(part 1 of 2)
# Autodesk Inventor assembly: 1000_Planar Winding Jig Overall Assembly_V1
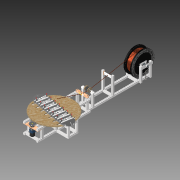
[picture p0: Inventor's stored thumbnail of the model, 180x180]
Saved by Autodesk Inventor 2020 (Build 240168000, 168)
## iProperties
Created: 2019-10-15
Part Number: 1000_Planar Winding Jig Overall Assembly_V1
Document SubType Name: Assembly
Designer: MPI
Author: MPI
## Documents named in this file (59)
- C:\Users\RFLab\Dropbox\MPI Group Folder\Winding Jigs\1000_Planar Winding Jig Overall Assembly_V1.iam
- C:\Users\RFLab\Dropbox\MPI Group Folder\Monika misc\inner winding jig\frame_1385mm.ipt
- C:\Users\RFLab\Dropbox\MPI Group Folder\Monika misc\inner winding jig\frame_1660mm.ipt
- C:\Users\RFLab\Dropbox\MPI Group Folder\Monika misc\inner winding jig\frame_300mm.ipt
- C:\Users\RFLab\Dropbox\MPI Group Folder\Monika misc\inner winding jig\frame_265mm.ipt
- C:\Users\RFLab\Dropbox\MPI Group Folder\Monika misc\inner winding jig\frame_215.5mm.ipt
- C:\Users\RFLab\Dropbox\MPI Group Folder\Monika misc\inner winding jig\frame_210mm.ipt
- C:\Users\RFLab\Dropbox\MPI Group Folder\Monika misc\inner winding jig\frame_275mm.ipt
- C:\Users\RFLab\Dropbox\MPI Group Folder\Monika misc\inner winding jig\frame_318mm.ipt
- C:\Users\RFLab\Dropbox\MPI Group Folder\Monika misc\inner winding jig\frame_440mm.ipt
- C:\Users\RFLab\Dropbox\MPI Group Folder\Monika misc\inner winding jig\frame_370mm.ipt
- C:\Users\RFLab\Dropbox\MPI Group Folder\Monika misc\inner winding jig\92991A190_BRASS CUP POINT SET SCREW.ipt
- C:\Users\RFLab\Dropbox\MPI Group Folder\Winding Jigs\1xxx_Planar Winding Jig\13xx_Winding Former\132x_Former Accessory\1321_Toggle Clamp_V1.ipt
- C:\Users\RFLab\Dropbox\MPI Group Folder\Winding Jigs\1xxx_Planar Winding Jig\13xx_Winding Former\132x_Former Accessory\1322_Clamp Holder_V1.ipt
- C:\Users\RFLab\Dropbox\MPI Group Folder\Winding Jigs\1xxx_Planar Winding Jig\13xx_Winding Former\132x_Former Accessory\1322a_Clamp Holder M4Bolt_V1.ipt
- C:\Users\RFLab\Dropbox\MPI Group Folder\Winding Jigs\1xxx_Planar Winding Jig\13xx_Winding Former\132x_Former Accessory\1323_Clamp Holder Pin_V1.ipt
- C:\Users\RFLab\Documents\Inventor\Content Center Files\R2020\en-US\AS 1474(1)\AS 1474 - M4(1).ipt
- C:\Users\RFLab\Dropbox\MPI Group Folder\Winding Jigs\1xxx_Planar Winding Jig\13xx_Winding Former\132x_Former Accessory\1324_Clamp Rail_V1.ipt
- C:\Users\RFLab\Dropbox\MPI Group Folder\Winding Jigs\1xxx_Planar Winding Jig\13xx_Winding Former\132x_Former Accessory\1325_Former Plate Bolts_V1.ipt
- C:\Users\RFLab\Dropbox\MPI Group Folder\Winding Jigs\1xxx_Planar Winding Jig\13xx_Winding Former\132x_Former Accessory\1326_Thumb Screw_V1.ipt
- C:\Users\RFLab\Dropbox\MPI Group Folder\Winding Jigs\1xxx_Planar Winding Jig\12xx_Non-Frame Structural\122x_Motor and Former Structure\1221_Center Former Shaft_V1.ipt
- C:\Users\RFLab\Dropbox\MPI Group Folder\Winding Jigs\1xxx_Planar Winding Jig\12xx_Non-Frame Structural\122x_Motor and Former Structure\1222_Former Shaft Plate_V1.ipt
- C:\Users\RFLab\Dropbox\MPI Group Folder\Winding Jigs\1xxx_Planar Winding Jig\12xx_Non-Frame Structural\122x_Motor and Former Structure\1223_Motor Plate_V1.ipt
- C:\Users\RFLab\Dropbox\MPI Group Folder\Winding Jigs\1xxx_Planar Winding Jig\12xx_Non-Frame Structural\122x_Motor and Former Structure\1225_Pinon_V1.ipt
- C:\Users\RFLab\Dropbox\MPI Group Folder\Winding Jigs\1xxx_Planar Winding Jig\12xx_Non-Frame Structural\122x_Motor and Former Structure\1225a_Pinion Collar_V1.ipt
- C:\Users\RFLab\Dropbox\MPI Group Folder\Winding Jigs\1xxx_Planar Winding Jig\12xx_Non-Frame Structural\122x_Motor and Former Structure\1226_Flat Head Screw_V1.ipt
- C:\Users\RFLab\Dropbox\MPI Group Folder\Winding Jigs\1xxx_Planar Winding Jig\12xx_Non-Frame Structural\122x_Motor and Former Structure\1224_Stepper Motor_V1.ipt
- C:\Users\RFLab\Dropbox\MPI Group Folder\Winding Jigs\1xxx_Planar Winding Jig\12xx_Non-Frame Structural\122x_Motor and Former Structure\1224a_Stepper Motor Gearbox_V1.ipt
- C:\Users\RFLab\Dropbox\MPI Group Folder\Winding Jigs\1xxx_Planar Winding Jig\13xx_Winding Former\131x_Former Plates\1312_Former Middle_V1.ipt
- C:\Users\RFLab\Dropbox\MPI Group Folder\Winding Jigs\1xxx_Planar Winding Jig\13xx_Winding Former\131x_Former Plates\1311_Former Top_V1.ipt
- C:\Users\RFLab\Dropbox\MPI Group Folder\Winding Jigs\1xxx_Planar Winding Jig\13xx_Winding Former\131x_Former Plates\1313_Former Bottom_V1.ipt
- C:\Users\RFLab\Dropbox\MPI Group Folder\Winding Jigs\1xxx_Planar Winding Jig\12xx_Non-Frame Structural\122x_Motor and Former Structure\1227_Former Shaft Bearing_V1.ipt
- C:\Users\RFLab\Dropbox\MPI Group Folder\Winding Jigs\1xxx_Planar Winding Jig\12xx_Non-Frame Structural\122x_Motor and Former Structure\1228_Major Gear_V1.ipt
- C:\Users\RFLab\Dropbox\MPI Group Folder\Winding Jigs\1xxx_Planar Winding Jig\12xx_Non-Frame Structural\121x_Wire Guidance\1211_Distal Roller Plate_V1.ipt
- C:\Users\RFLab\Dropbox\MPI Group Folder\Winding Jigs\1xxx_Planar Winding Jig\12xx_Non-Frame Structural\121x_Wire Guidance\1212_Roller Plate Bolt_V1.ipt
- C:\Users\RFLab\Dropbox\MPI Group Folder\Winding Jigs\1xxx_Planar Winding Jig\12xx_Non-Frame Structural\121x_Wire Guidance\1213_Distal Roller_V1.ipt
- C:\Users\RFLab\Dropbox\MPI Group Folder\Winding Jigs\1xxx_Planar Winding Jig\12xx_Non-Frame Structural\121x_Wire Guidance\1214_Shaft Collar 3-16_V1.ipt
- C:\Users\RFLab\Dropbox\MPI Group Folder\Winding Jigs\1xxx_Planar Winding Jig\12xx_Non-Frame Structural\121x_Wire Guidance\1215_3-8 Roller Shaft_V1.ipt
- C:\Users\RFLab\Dropbox\MPI Group Folder\Winding Jigs\1xxx_Planar Winding Jig\12xx_Non-Frame Structural\121x_Wire Guidance\1216_Roller Spacer_V1.ipt
- C:\Users\RFLab\Dropbox\MPI Group Folder\Winding Jigs\1xxx_Planar Winding Jig\12xx_Non-Frame Structural\121x_Wire Guidance\1217_17mm Shaft_V1.ipt
- C:\Users\RFLab\Dropbox\MPI Group Folder\Winding Jigs\1xxx_Planar Winding Jig\12xx_Non-Frame Structural\121x_Wire Guidance\1218_Angular Contact Bearing 17mm_V1.ipt
- C:\Users\RFLab\Dropbox\MPI Group Folder\Winding Jigs\1xxx_Planar Winding Jig\12xx_Non-Frame Structural\121x_Wire Guidance\1219_Middle Roller_V1.ipt
- C:\Users\RFLab\Dropbox\MPI Group Folder\Winding Jigs\1xxx_Planar Winding Jig\12xx_Non-Frame Structural\121x_Wire Guidance\12110_Shaft Cap_V1.ipt
- C:\Users\RFLab\Dropbox\MPI Group Folder\Winding Jigs\1xxx_Planar Winding Jig\12xx_Non-Frame Structural\121x_Wire Guidance\12111_Proximal Roller_V1.ipt
- C:\Users\RFLab\Dropbox\MPI Group Folder\Winding Jigs\1xxx_Planar Winding Jig\12xx_Non-Frame Structural\121x_Wire Guidance\12112_Proximal Roller Plate_V1.ipt
- C:\Users\RFLab\Dropbox\MPI Group Folder\Winding Jigs\1xxx_Planar Winding Jig\12xx_Non-Frame Structural\121x_Wire Guidance\12113_Proximal Roller Shaft_V1.ipt
- C:\Users\RFLab\Dropbox\MPI Group Folder\Winding Jigs\1xxx_Planar Winding Jig\12xx_Non-Frame Structural\121x_Wire Guidance\12114_3-8 Shaft Bearing_V1.ipt
- C:\Users\RFLab\Dropbox\MPI Group Folder\Winding Jigs\1xxx_Planar Winding Jig\12xx_Non-Frame Structural\123x_Spool Holder\1231_Spool Shaft_V1.ipt
- C:\Users\RFLab\Dropbox\MPI Group Folder\Winding Jigs\1xxx_Planar Winding Jig\12xx_Non-Frame Structural\123x_Spool Holder\1233_Spool Holding Bolts_V1.ipt
- C:\Users\RFLab\Dropbox\MPI Group Folder\Winding Jigs\1xxx_Planar Winding Jig\12xx_Non-Frame Structural\123x_Spool Holder\1232_Spool Shaft Collar_V1.ipt
- C:\Users\RFLab\Dropbox\MPI Group Folder\Winding Jigs\1xxx_Planar Winding Jig\12xx_Non-Frame Structural\123x_Spool Holder\1234_Spool Plate_V1.ipt
- C:\Users\RFLab\Dropbox\MPI Group Folder\Winding Jigs\1xxx_Planar Winding Jig\12xx_Non-Frame Structural\123x_Spool Holder\1235_Shaft Locking Screw_V1.ipt
- C:\Users\RFLab\Dropbox\MPI Group Folder\Winding Jigs\1xxx_Planar Winding Jig\12xx_Non-Frame Structural\123x_Spool Holder\1236_Spool Shaft Support Plate_V1.ipt
- C:\Users\RFLab\Dropbox\MPI Group Folder\Winding Jigs\1xxx_Planar Winding Jig\12xx_Non-Frame Structural\123x_Spool Holder\1237_Turnbuckle_V1.ipt
- C:\Users\RFLab\Dropbox\MPI Group Folder\Winding Jigs\1xxx_Planar Winding Jig\12xx_Non-Frame Structural\123x_Spool Holder\1238_Hex Nut Turnbuckle_V1.ipt
- C:\Users\RFLab\Dropbox\MPI Group Folder\Winding Jigs\1xxx_Planar Winding Jig\12xx_Non-Frame Structural\123x_Spool Holder\1239_Turnbuckle Holding Bolt_V1.ipt
- C:\Users\RFLab\Dropbox\MPI Group Folder\Winding Jigs\1xxx_Planar Winding Jig\12xx_Non-Frame Structural\123x_Spool Holder\12310_Washer_V1.ipt
- C:\Users\RFLab\Dropbox\MPI Group Folder\Winding Jigs\1xxx_Planar Winding Jig\12xx_Non-Frame Structural\1240_Wire Spool and Wire.ipt
- C:\Users\RFLab\Dropbox\MPI Group Folder\Winding Jigs\1xxx_Planar Winding Jig\12xx_Non-Frame Structural\1240x_Wire Depiction_V1.ipt
## Components (321 placed, 58 different names)
1. 1222_Former Shaft Plate_V1:1 — Mate:46, Flush:77, Mate:47, Insert:1
2. 1222_Former Shaft Plate_V1:2 — Mate:48, Flush:78, Mate:49
3. 1221_Center Former Shaft_V1:1 — Insert:1, Mate:51, Mate:53, Mate:55, Mate:57
4. 1228_Major Gear_V1:1 — Mate:50, Mate:51, Insert:2, Mate:52, Insert:3, Insert:4, Insert:5, Insert:6, Insert:7, Insert:8, Insert:9, Insert:10, Insert:11, Insert:12, Insert:13, Insert:14, Insert:15, Insert:16, Flush:84
5. 1227_Former Shaft Bearing_V1:1 — Insert:2
6. 1224a_Stepper Motor Gearbox_V1:1 — Insert:38, Insert:39, Insert:40, Insert:41, Mate:65
7. 1224_Stepper Motor_V1:1 — Insert:40, Insert:41
8. 1225_Pinon_V1:1 — Flush:84, Mate:64, Insert:42, Insert:43
9. 1225a_Pinion Collar_V1:1 — Mate:64, Mate:65, Insert:42, Insert:43, Angle:36
10. 1211_Distal Roller Plate_V1:1 — Insert:46, Insert:47, Flush:87, Flush:88, Insert:50, Insert:51, Insert:58, Insert:59, Mate:70, Mate:72
11. 1213_Distal Roller_V1:1 — Insert:44, Insert:46, Insert:48
12. 1213_Distal Roller_V1:2 — Insert:45, Insert:47, Insert:49, Mate:68, Flush:294
13. 12114_3-8 Shaft Bearing_V1:1 — Insert:44
14. 12114_3-8 Shaft Bearing_V1:2 — Insert:45
15. 12114_3-8 Shaft Bearing_V1:3 — Insert:48
16. 12114_3-8 Shaft Bearing_V1:4 — Insert:49
17. 1211_Distal Roller Plate_V1:2 — Mate:68, Flush:87, Flush:88, Insert:52, Insert:53, Insert:54, Insert:55, Insert:56, Insert:57
18. 1216_Roller Spacer_V1:1 — Insert:51
19. 1216_Roller Spacer_V1:2 — Insert:50
20. 1212_Roller Plate Bolt_V1:1 — Insert:52
21. 1212_Roller Plate Bolt_V1:2 — Insert:53
22. 1215_3-8 Roller Shaft_V1:1 — Insert:54
23. 1215_3-8 Roller Shaft_V1:2 — Insert:55
24. 1214_Shaft Collar 3-16_V1:1 — Insert:58
25. 1214_Shaft Collar 3-16_V1:2 — Insert:59
26. 1214_Shaft Collar 3-16_V1:3 — Insert:56
27. 1214_Shaft Collar 3-16_V1:4 — Insert:57
28. 12110_Shaft Cap_V1:1 — Mate:75, Mate:76, Mate:77
29. 12110_Shaft Cap_V1:2 — Mate:78, Mate:79, Mate:80, Insert:60, Insert:61
30. 1219_Middle Roller_V1:1 — Insert:61, Insert:62, Insert:63, Flush:292
31. 1217_17mm Shaft_V1:1 — Insert:60
32. 1218_Angular Contact Bearing 17mm_V1:1 — Insert:62
33. 1218_Angular Contact Bearing 17mm_V1:2 — Insert:63
34. frame_440mm:1 — Mate:81, Flush:97, Flush:98, Mate:84, Flush:103, Flush:104
35. frame_440mm:2 — Mate:82, Flush:99, Flush:100, Mate:83, Flush:101, Flush:102
36. 12112_Proximal Roller Plate_V1:1 — Mate:83, Flush:101, Flush:102, Insert:74, Insert:75
37. 12112_Proximal Roller Plate_V1:2 — Mate:84, Flush:103, Flush:104, Insert:64, Insert:65, Insert:70, Insert:71, Insert:72, Insert:73
38. 12113_Proximal Roller Shaft_V1:1 — Insert:64
39. 12113_Proximal Roller Shaft_V1:2 — Insert:65
40. 12111_Proximal Roller_V1:1 — Insert:66, Insert:68, Insert:70
41. 12111_Proximal Roller_V1:2 — Insert:67, Insert:69, Insert:71
42. 12114_3-8 Shaft Bearing_V1:5 — Insert:66
43. 12114_3-8 Shaft Bearing_V1:6 — Insert:68
44. 12114_3-8 Shaft Bearing_V1:7 — Insert:67
45. 12114_3-8 Shaft Bearing_V1:8 — Insert:69
46. 1236_Spool Shaft Support Plate_V1:1 — Mate:90, Flush:114, Flush:115, Flush:116, Insert:76, Insert:77, Angle:37
47. 1236_Spool Shaft Support Plate_V1:2 — Mate:89, Flush:111, Flush:112, Flush:113, Insert:78, Angle:1
48. 92991A190_BRASS CUP POINT SET SCREW:1 — Insert:73
49. 92991A190_BRASS CUP POINT SET SCREW:2 — Insert:72
50. 92991A190_BRASS CUP POINT SET SCREW:3 — Insert:75
51. 92991A190_BRASS CUP POINT SET SCREW:4 — Insert:74
52. 1231_Spool Shaft_V1:1 — Insert:76, Angle:1, Mate:354, Mate:360
53. 1232_Spool Shaft Collar_V1:1 — Insert:77
54. 1232_Spool Shaft Collar_V1:2 — Insert:78
55. 1240_Wire Spool and Wire:1 — Mate:354, Mate:355, Mate:356, Angle:34, Flush:292, Mate:357, Mate:358, Mate:359
56. 1234_Spool Plate_V1:1 — Insert:84, Insert:85, Insert:86, Mate:355, Flush:293, Angle:37, Flush:295, Flush:296, Mate:360
57. 1234_Spool Plate_V1:2 — Insert:82, Insert:83, Insert:87, Mate:356, Angle:34, Flush:293, Flush:295, Flush:296
58. 1233_Spool Holding Bolts_V1:1 — Insert:82
59. 1233_Spool Holding Bolts_V1:2 — Insert:83
60. 1233_Spool Holding Bolts_V1:3 — Insert:84
61. 1233_Spool Holding Bolts_V1:4 — Insert:85
62. 1235_Shaft Locking Screw_V1:1 — Insert:86
63. 1235_Shaft Locking Screw_V1:2 — Insert:87
64. 12310_Washer_V1:1 — Insert:88, Insert:91
65. 12310_Washer_V1:2 — Insert:89, Insert:90
66. 1239_Turnbuckle Holding Bolt_V1:1 — Insert:91, Mate:91, Insert:98
67. 1239_Turnbuckle Holding Bolt_V1:2 — Insert:90, Mate:92, Insert:99
68. 12310_Washer_V1:3 — Insert:92, Insert:96
69. 12310_Washer_V1:4 — Insert:93, Insert:94
70. 1238_Hex Nut Turnbuckle_V1:1 — Insert:94, Insert:95
71. 1238_Hex Nut Turnbuckle_V1:2 — Insert:95
72. 1238_Hex Nut Turnbuckle_V1:3 — Insert:96, Insert:97
73. 1238_Hex Nut Turnbuckle_V1:4 — Insert:97
74. 1237_Turnbuckle_V1:1 — Mate:91, Angle:3
75. 1237_Turnbuckle_V1:2 — Mate:92, Angle:4
76. 1238_Hex Nut Turnbuckle_V1:5 — Insert:98
77. 1238_Hex Nut Turnbuckle_V1:6 — Insert:99
78. 1240x_Wire Depiction_V1:1 — Mate:357, Mate:358, Angle:35, Mate:359, Flush:294
79. frame_318mm:2 — Mate:74, Flush:95, Flush:96, Mate:75, Mate:76, Mate:77
80. frame_318mm:1 — Mate:73, Flush:93, Flush:94, Mate:78, Mate:79, Mate:80
81. frame_275mm:2 — Mate:71, Mate:72, Flush:91, Flush:92
82. frame_275mm:1 — Mate:69, Mate:70, Flush:89, Flush:90
83. frame_370mm:4 — Flush:107, Mate:86, Flush:116, Angle:4
84. frame_370mm:3 — Flush:105, Flush:106, Mate:85, Mate:90, Flush:114, Flush:115
85. frame_370mm:2 — Mate:88, Flush:110, Flush:113, Angle:3
86. frame_370mm:1 — Mate:87, Flush:108, Flush:109, Mate:89, Flush:111, Flush:112
87. frame_1385mm:1 — Mate:1, Flush:1, Mate:2, Flush:2, Flush:3, Mate:3, Mate:9, Mate:10, Flush:18, Mate:14, Flush:20, Mate:15, Mate:22, Flush:34, Mate:23, Flush:36, Mate:24, Flush:38, Flush:46, Flush:47, Flush:67, Mate:38, Mate:39
88. frame_1385mm:2 — Flush:2, Flush:3, Mate:3, Flush:4, Mate:4, Mate:5, Flush:6, Mate:8, Flush:7, Flush:8, Flush:9, Flush:10, Flush:11, Flush:12, Mate:11, Flush:13, Flush:14, Mate:12, Flush:15, Mate:19, Flush:28, Mate:20, Flush:30, Mate:21, Flush:32, Flush:33, Flush:44, Flush:45, Mate:47
89. frame_1660mm:2 — Flush:4, Mate:4, Mate:5, Flush:66, Flush:74, Mate:69, Flush:90, Mate:74, Flush:96, Mate:82, Flush:99, Mate:87, Mate:88, Flush:108, Flush:109, Flush:110, Insert:88, Insert:92
90. frame_300mm:1 — Flush:6, Mate:8, Flush:7
91. frame_300mm:2 — Flush:8, Mate:9, Flush:9, Flush:61, Mate:46, Flush:77
92. frame_300mm:3 — Flush:10, Mate:10, Flush:11, Flush:63
93. frame_265mm:1 — Flush:12, Mate:11, Flush:13, Mate:13, Flush:17, Flush:19, Flush:29
94. frame_265mm:2 — Flush:14, Mate:12, Flush:15, Flush:16, Flush:21, Flush:31
95. frame_265mm:3 — Flush:16, Mate:13, Flush:17, Mate:17, Flush:24, Flush:25, Mate:18, Flush:26, Flush:27
96. frame_265mm:4 — Flush:18, Mate:14, Flush:19, Flush:22, Mate:16, Flush:23, Flush:37
97. frame_265mm:5 — Flush:20, Mate:15, Flush:21, Flush:39, Flush:42
98. frame_265mm:6 — Flush:22, Mate:16, Flush:23, Mate:25, Flush:40, Flush:41, Mate:26, Flush:43
99. frame_215.5mm:1 — Mate:19, Flush:28, Flush:29
100. frame_215.5mm:2 — Mate:20, Flush:30, Flush:31
101. frame_215.5mm:3 — Mate:17, Flush:24, Flush:25
102. frame_215.5mm:4 — Mate:18, Flush:26, Flush:27, Mate:32, Flush:54, Flush:55
103. frame_215.5mm:5 — Mate:21, Flush:32, Flush:33, Flush:35, Mate:27
104. frame_215.5mm:6 — Mate:25, Flush:40, Flush:41, Mate:29, Flush:48, Flush:49
105. frame_215.5mm:7 — Mate:24, Flush:38, Flush:39
106. frame_215.5mm:8 — Mate:22, Flush:34, Flush:35, Mate:28
107. frame_215.5mm:9 — Mate:23, Flush:36, Flush:37
108. frame_215.5mm:10 — Mate:26, Flush:42, Flush:43
109. frame_1385mm:3 — Mate:27, Flush:44, Flush:45, Mate:33, Mate:34, Mate:49, Mate:63, Flush:82, Flush:83
110. frame_1385mm:4 — Mate:28, Flush:46, Flush:47, Mate:30, Mate:31, Mate:35, Flush:60, Mate:36, Flush:62, Mate:50, Angle:9, Angle:36
111. frame_265mm:7 — Mate:29, Flush:48, Flush:49, Flush:50, Flush:51, Flush:52, Flush:53
112. frame_265mm:8 — Mate:31, Flush:52, Flush:53
113. frame_265mm:9 — Mate:32, Flush:54, Flush:55, Flush:56, Flush:57, Flush:58, Flush:59
114. frame_265mm:10 — Mate:30, Flush:50, Flush:51
115. frame_265mm:11 — Mate:34, Flush:58, Flush:59
116. frame_265mm:12 — Mate:33, Flush:56, Flush:57
117. frame_300mm:4 — Mate:35, Flush:60, Flush:61, Mate:48, Flush:78
118. frame_300mm:5 — Mate:36, Flush:62, Flush:63
119. frame_210mm:1 — Mate:40, Flush:68, Flush:69, Mate:43, Flush:76, Flush:89, Flush:91
120. frame_210mm:2 — Mate:42, Flush:72, Mate:43, Flush:93, Flush:95
121. frame_210mm:3 — Mate:44, Flush:73, Flush:74, Flush:98, Flush:100
122. frame_210mm:4 — Mate:45, Flush:75, Flush:76
123. frame_1660mm:3 — Flush:66, Flush:67, Mate:38, Mate:39, Mate:40, Flush:68, Flush:69, Mate:42, Flush:72, Mate:44, Flush:73, Mate:45, Flush:75, Mate:71, Flush:92, Mate:73, Flush:94, Mate:81, Flush:97, Flush:105, Flush:106, Mate:85, Flush:107, Mate:86, Insert:89, Insert:93
124. 1325_Former Plate Bolts_V1:1 — Insert:100
125. 1325_Former Plate Bolts_V1:2 — Insert:101
126. 1325_Former Plate Bolts_V1:3 — Insert:102
127. 1325_Former Plate Bolts_V1:4 — Insert:103
128. 1325_Former Plate Bolts_V1:5 — Insert:104
129. 1325_Former Plate Bolts_V1:6 — Insert:105
130. 1325_Former Plate Bolts_V1:7 — Insert:106
131. 1325_Former Plate Bolts_V1:8 — Insert:107
132. 1325_Former Plate Bolts_V1:9 — Insert:108
133. 1325_Former Plate Bolts_V1:10 — Insert:109
134. 1325_Former Plate Bolts_V1:11 — Insert:110
135. 1325_Former Plate Bolts_V1:12 — Insert:111
136. 1313_Former Bottom_V1:1 — Mate:52, Mate:53, Insert:3, Insert:4, Mate:54, Insert:17, Angle:9
137. 1226_Flat Head Screw_V1:1 — Insert:10
138. 1226_Flat Head Screw_V1:2 — Insert:14
139. 1226_Flat Head Screw_V1:3 — Insert:15
140. 1226_Flat Head Screw_V1:4 — Insert:7
141. 1226_Flat Head Screw_V1:5 — Insert:11
142. 1226_Flat Head Screw_V1:6 — Insert:12
143. 1226_Flat Head Screw_V1:7 — Insert:13
144. 1226_Flat Head Screw_V1:8 — Insert:5
145. 1226_Flat Head Screw_V1:9 — Insert:16
146. 1226_Flat Head Screw_V1:10 — Insert:9
147. 1226_Flat Head Screw_V1:11 — Insert:8
148. 1226_Flat Head Screw_V1:12 — Insert:6
149. 1312_Former Middle_V1:1 — Mate:54, Mate:55, Insert:17, Mate:56, Insert:18
150. 1311_Former Top_V1:1 — Mate:56, Mate:57, Insert:18, Mate:58, Insert:31, Insert:32, Mate:59, Insert:33, Insert:34, Mate:60, Insert:35, Insert:36, Insert:37, Insert:100, Insert:101, Insert:102, Insert:103, Insert:104, Insert:105, Insert:106, Insert:107, Insert:108, Insert:109, Insert:110, Insert:111, Mate:122, Flush:134, Mate:160, Mate:163, Mate:164, Flush:160, Mate:201, Mate:202, Mate:203, Mate:348, Mate:349, Mate:350, Mate:351, Mate:352, Mate:353
151. 1326_Thumb Screw_V1:1 — Insert:37
152. 1326_Thumb Screw_V1:2 — Insert:36
153. 1223_Motor Plate_V1:1 — Mate:63, Flush:82, Flush:83, Insert:38, Insert:39
154. 1324_Clamp Rail_V1:1 — Mate:58, Insert:31, Insert:32, Flush:79
155. 1324_Clamp Rail_V1:2 — Mate:59, Insert:33, Insert:34, Mate:61, Mate:123, Flush:135
156. 1322_Clamp Holder_V1:1 — Mate:60, Flush:79, Mate:61, Mate:62, Flush:80, Flush:81, Mate:93, Mate:94, Angle:5, Mate:95, Mate:96, Angle:6, Mate:97, Mate:98, Mate:99, Mate:125
157. 1321_Toggle Clamp_V1:1 — Mate:62, Flush:80, Flush:81, Mate:101, Mate:103, Mate:105
158. 1323_Clamp Holder Pin_V1:1 — Insert:35, Mate:125
159. BS 3692 Precision hexagon bolts and screws (Full Threaded) - Metric M4 x 9:1 — Mate:95, Mate:96, Angle:6, Flush:119, Mate:100
160. BS 3692 Precision hexagon bolts and screws (Full Threaded) - Metric M4 x 9:2 — Mate:93, Mate:94, Angle:5, Flush:120, Mate:106
161. BS 3692 Precision hexagon bolts and screws (Full Threaded) - Metric M4 x 9:3 — Flush:118, Mate:99, Flush:120, Mate:104
162. BS 3692 Precision hexagon bolts and screws (Full Threaded) - Metric M4 x 9:4 — Flush:118, Mate:97, Mate:98, Flush:119, Mate:102
163. AS 1474 - Metric M4:1 — Mate:100, Mate:101, Flush:124
164. AS 1474 - Metric M4:2 — Flush:121, Flush:123, Mate:102, Mate:103
165. AS 1474 - Metric M4:3 — Flush:122, Flush:123, Mate:104
166. AS 1474 - Metric M4:4 — Flush:121, Flush:122, Mate:105, Mate:106, Flush:124
167. 1322_Clamp Holder_V1:2 — Mate:122, Mate:123, Mate:124, Flush:135
168. 1321_Toggle Clamp_V1:2
169. 1323_Clamp Holder Pin_V1:2 — Flush:134, Mate:124, Flush:185
170. BS 3692 Precision hexagon bolts and screws (Full Threaded) - Metric M4 x 9:5
171. BS 3692 Precision hexagon bolts and screws (Full Threaded) - Metric M4 x 9:6
172. BS 3692 Precision hexagon bolts and screws (Full Threaded) - Metric M4 x 9:7
173. BS 3692 Precision hexagon bolts and screws (Full Threaded) - Metric M4 x 9:8
174. AS 1474 - Metric M4:5
175. AS 1474 - Metric M4:6
176. AS 1474 - Metric M4:7
177. AS 1474 - Metric M4:8
178. 1324_Clamp Rail_V1:3 — Mate:160, Flush:156, Mate:162, Flush:158
179. 1324_Clamp Rail_V1:4 — Flush:156, Mate:161, Mate:163, Mate:164, Flush:158
180. 1322_Clamp Holder_V1:3 — Mate:161, Flush:157
181. 1321_Toggle Clamp_V1:3
182. 1323_Clamp Holder Pin_V1:3 — Flush:159
183. BS 3692 Precision hexagon bolts and screws (Full Threaded) - Metric M4 x 9:9
184. BS 3692 Precision hexagon bolts and screws (Full Threaded) - Metric M4 x 9:10
185. BS 3692 Precision hexagon bolts and screws (Full Threaded) - Metric M4 x 9:11
186. BS 3692 Precision hexagon bolts and screws (Full Threaded) - Metric M4 x 9:12
187. AS 1474 - Metric M4:9
188. AS 1474 - Metric M4:10
189. AS 1474 - Metric M4:11
190. AS 1474 - Metric M4:12
191. 1322_Clamp Holder_V1:4 — Flush:157, Mate:162
192. 1321_Toggle Clamp_V1:4
193. 1323_Clamp Holder Pin_V1:4 — Flush:159, Flush:160, Flush:291
194. BS 3692 Precision hexagon bolts and screws (Full Threaded) - Metric M4 x 9:13
195. BS 3692 Precision hexagon bolts and screws (Full Threaded) - Metric M4 x 9:14
196. BS 3692 Precision hexagon bolts and screws (Full Threaded) - Metric M4 x 9:15
197. BS 3692 Precision hexagon bolts and screws (Full Threaded) - Metric M4 x 9:16
198. AS 1474 - Metric M4:13
199. AS 1474 - Metric M4:14
200. AS 1474 - Metric M4:15
201. AS 1474 - Metric M4:16
202. 1324_Clamp Rail_V1:5
203. 1324_Clamp Rail_V1:6 — Mate:201, Mate:202, Mate:203
204. 1322_Clamp Holder_V1:5
205. 1321_Toggle Clamp_V1:5
206. 1323_Clamp Holder Pin_V1:5
207. BS 3692 Precision hexagon bolts and screws (Full Threaded) - Metric M4 x 9:17
208. BS 3692 Precision hexagon bolts and screws (Full Threaded) - Metric M4 x 9:18
209. BS 3692 Precision hexagon bolts and screws (Full Threaded) - Metric M4 x 9:19
210. BS 3692 Precision hexagon bolts and screws (Full Threaded) - Metric M4 x 9:20
211. AS 1474 - Metric M4:17
212. AS 1474 - Metric M4:18
213. AS 1474 - Metric M4:19
214. AS 1474 - Metric M4:20
215. 1322_Clamp Holder_V1:6
216. 1321_Toggle Clamp_V1:6
217. 1323_Clamp Holder Pin_V1:6 — Flush:185
218. BS 3692 Precision hexagon bolts and screws (Full Threaded) - Metric M4 x 9:21
219. BS 3692 Precision hexagon bolts and screws (Full Threaded) - Metric M4 x 9:22
220. BS 3692 Precision hexagon bolts and screws (Full Threaded) - Metric M4 x 9:23
221. BS 3692 Precision hexagon bolts and screws (Full Threaded) - Metric M4 x 9:24
222. AS 1474 - Metric M4:21
223. AS 1474 - Metric M4:22
224. AS 1474 - Metric M4:23
225. AS 1474 - Metric M4:24
226. 1324_Clamp Rail_V1:7 — Flush:282, Flush:285
227. 1324_Clamp Rail_V1:8 — Mate:348, Mate:349, Mate:350
228. 1322_Clamp Holder_V1:7
229. 1321_Toggle Clamp_V1:7
230. 1323_Clamp Holder Pin_V1:7
231. BS 3692 Precision hexagon bolts and screws (Full Threaded) - Metric M4 x 9:25
232. BS 3692 Precision hexagon bolts and screws (Full Threaded) - Metric M4 x 9:26
233. BS 3692 Precision hexagon bolts and screws (Full Threaded) - Metric M4 x 9:27
234. BS 3692 Precision hexagon bolts and screws (Full Threaded) - Metric M4 x 9:28
235. AS 1474 - Metric M4:25
236. AS 1474 - Metric M4:26
237. AS 1474 - Metric M4:27
238. AS 1474 - Metric M4:28
239. 1322_Clamp Holder_V1:8
240. 1321_Toggle Clamp_V1:8
241. 1323_Clamp Holder Pin_V1:8 — Flush:288, Flush:291
242. BS 3692 Precision hexagon bolts and screws (Full Threaded) - Metric M4 x 9:29
243. BS 3692 Precision hexagon bolts and screws (Full Threaded) - Metric M4 x 9:30
244. BS 3692 Precision hexagon bolts and screws (Full Threaded) - Metric M4 x 9:31
245. BS 3692 Precision hexagon bolts and screws (Full Threaded) - Metric M4 x 9:32
246. AS 1474 - Metric M4:29
247. AS 1474 - Metric M4:30
248. AS 1474 - Metric M4:31
249. AS 1474 - Metric M4:32
250. 1324_Clamp Rail_V1:9 — Flush:286, Mate:351
251. 1324_Clamp Rail_V1:10 — Flush:282, Flush:283, Flush:285
252. 1322_Clamp Holder_V1:9
253. 1321_Toggle Clamp_V1:9
254. 1323_Clamp Holder Pin_V1:9
255. BS 3692 Precision hexagon bolts and screws (Full Threaded) - Metric M4 x 9:33
256. BS 3692 Precision hexagon bolts and screws (Full Threaded) - Metric M4 x 9:34
257. BS 3692 Precision hexagon bolts and screws (Full Threaded) - Metric M4 x 9:35
258. BS 3692 Precision hexagon bolts and screws (Full Threaded) - Metric M4 x 9:36
259. AS 1474 - Metric M4:33
260. AS 1474 - Metric M4:34
261. AS 1474 - Metric M4:35
262. AS 1474 - Metric M4:36
263. 1322_Clamp Holder_V1:10
264. 1321_Toggle Clamp_V1:10
265. 1323_Clamp Holder Pin_V1:10 — Flush:288, Flush:289
266. BS 3692 Precision hexagon bolts and screws (Full Threaded) - Metric M4 x 9:37
267. BS 3692 Precision hexagon bolts and screws (Full Threaded) - Metric M4 x 9:38
268. BS 3692 Precision hexagon bolts and screws (Full Threaded) - Metric M4 x 9:39
269. BS 3692 Precision hexagon bolts and screws (Full Threaded) - Metric M4 x 9:40
270. AS 1474 - Metric M4:37
271. AS 1474 - Metric M4:38
272. AS 1474 - Metric M4:39
273. AS 1474 - Metric M4:40
274. 1324_Clamp Rail_V1:11 — Flush:284, Flush:287
275. 1324_Clamp Rail_V1:12 — Flush:283, Flush:286, Mate:352
276. 1322_Clamp Holder_V1:11
277. 1321_Toggle Clamp_V1:11
278. 1323_Clamp Holder Pin_V1:11
279. BS 3692 Precision hexagon bolts and screws (Full Threaded) - Metric M4 x 9:41
280. BS 3692 Precision hexagon bolts and screws (Full Threaded) - Metric M4 x 9:42
281. BS 3692 Precision hexagon bolts and screws (Full Threaded) - Metric M4 x 9:43
282. BS 3692 Precision hexagon bolts and screws (Full Threaded) - Metric M4 x 9:44
283. AS 1474 - Metric M4:41
284. AS 1474 - Metric M4:42
285. AS 1474 - Metric M4:43
286. AS 1474 - Metric M4:44
287. 1322_Clamp Holder_V1:12
288. 1321_Toggle Clamp_V1:12
289. 1323_Clamp Holder Pin_V1:12 — Flush:289, Flush:290
290. BS 3692 Precision hexagon bolts and screws (Full Threaded) - Metric M4 x 9:45
291. BS 3692 Precision hexagon bolts and screws (Full Threaded) - Metric M4 x 9:46
292. BS 3692 Precision hexagon bolts and screws (Full Threaded) - Metric M4 x 9:47
293. BS 3692 Precision hexagon bolts and screws (Full Threaded) - Metric M4 x 9:48
294. AS 1474 - Metric M4:45
295. AS 1474 - Metric M4:46
296. AS 1474 - Metric M4:47
297. AS 1474 - Metric M4:48
298. 1324_Clamp Rail_V1:13
299. 1324_Clamp Rail_V1:14 — Flush:284, Flush:287, Mate:353
300. 1322_Clamp Holder_V1:13
301. 1321_Toggle Clamp_V1:13
302. 1323_Clamp Holder Pin_V1:13
303. BS 3692 Precision hexagon bolts and screws (Full Threaded) - Metric M4 x 9:49
304. BS 3692 Precision hexagon bolts and screws (Full Threaded) - Metric M4 x 9:50
305. BS 3692 Precision hexagon bolts and screws (Full Threaded) - Metric M4 x 9:51
306. BS 3692 Precision hexagon bolts and screws (Full Threaded) - Metric M4 x 9:52
307. AS 1474 - Metric M4:49
308. AS 1474 - Metric M4:50
309. AS 1474 - Metric M4:51
310. AS 1474 - Metric M4:52
311. 1322_Clamp Holder_V1:14
312. 1321_Toggle Clamp_V1:14
313. 1323_Clamp Holder Pin_V1:14 — Flush:290
314. BS 3692 Precision hexagon bolts and screws (Full Threaded) - Metric M4 x 9:53
315. BS 3692 Precision hexagon bolts and screws (Full Threaded) - Metric M4 x 9:54
316. BS 3692 Precision hexagon bolts and screws (Full Threaded) - Metric M4 x 9:55
317. BS 3692 Precision hexagon bolts and screws (Full Threaded) - Metric M4 x 9:56
318. AS 1474 - Metric M4:53
319. AS 1474 - Metric M4:54
320. AS 1474 - Metric M4:55
321. AS 1474 - Metric M4:56
## Relationships (774: Mate 354, Flush 288, Insert 96, Angle 36)
- Mate:1: frame_1385mm:1
- Flush:1: frame_1385mm:1
- Mate:2: frame_1385mm:1
- Flush:2: frame_1385mm:1 ↔ frame_1385mm:2
- Flush:3: frame_1385mm:1 ↔ frame_1385mm:2
- Mate:3 (300 mm): frame_1385mm:1 ↔ frame_1385mm:2
- Flush:4: frame_1385mm:2 ↔ frame_1660mm:2
- Mate:4: frame_1385mm:2 ↔ frame_1660mm:2
- Mate:5 (-45 mm): frame_1385mm:2 ↔ frame_1660mm:2
- Flush:6: frame_1385mm:2 ↔ frame_300mm:1
- Mate:8: frame_1385mm:2 ↔ frame_300mm:1
- Flush:7 (27 mm): frame_1385mm:2 ↔ frame_300mm:1
- Flush:8: frame_1385mm:2 ↔ frame_300mm:2
- Mate:9: frame_1385mm:1 ↔ frame_300mm:2
- Flush:9 (537 mm): frame_1385mm:2 ↔ frame_300mm:2
- Flush:10: frame_1385mm:2 ↔ frame_300mm:3
- Mate:10: frame_1385mm:1 ↔ frame_300mm:3
- Flush:11 (657 mm): frame_1385mm:2 ↔ frame_300mm:3
- Flush:12: frame_1385mm:2 ↔ frame_265mm:1
- Mate:11: frame_1385mm:2 ↔ frame_265mm:1
- Flush:13 (487 mm): frame_1385mm:2 ↔ frame_265mm:1
- Flush:14: frame_1385mm:2 ↔ frame_265mm:2
- Mate:12: frame_1385mm:2 ↔ frame_265mm:2
- Flush:15 (707 mm): frame_1385mm:2 ↔ frame_265mm:2
- Flush:16: frame_265mm:2 ↔ frame_265mm:3
- Mate:13: frame_265mm:1 ↔ frame_265mm:3
- Flush:17: frame_265mm:1 ↔ frame_265mm:3
- Flush:18: frame_1385mm:1 ↔ frame_265mm:4
- Mate:14: frame_1385mm:1 ↔ frame_265mm:4
- Flush:19: frame_265mm:1 ↔ frame_265mm:4
- Flush:20: frame_1385mm:1 ↔ frame_265mm:5
- Mate:15: frame_1385mm:1 ↔ frame_265mm:5
- Flush:21: frame_265mm:2 ↔ frame_265mm:5
- Flush:22: frame_265mm:4 ↔ frame_265mm:6
- Mate:16: frame_265mm:4 ↔ frame_265mm:6
- Flush:23: frame_265mm:4 ↔ frame_265mm:6
- Mate:17: frame_265mm:3 ↔ frame_215.5mm:3
- Flush:24: frame_265mm:3 ↔ frame_215.5mm:3
- Flush:25: frame_265mm:3 ↔ frame_215.5mm:3
- Mate:18: frame_265mm:3 ↔ frame_215.5mm:4
- Flush:26: frame_265mm:3 ↔ frame_215.5mm:4
- Flush:27: frame_265mm:3 ↔ frame_215.5mm:4
- Mate:19: frame_1385mm:2 ↔ frame_215.5mm:1
- Flush:28: frame_1385mm:2 ↔ frame_215.5mm:1
- Flush:29: frame_265mm:1 ↔ frame_215.5mm:1
- Mate:20: frame_1385mm:2 ↔ frame_215.5mm:2
- Flush:30: frame_1385mm:2 ↔ frame_215.5mm:2
- Flush:31: frame_265mm:2 ↔ frame_215.5mm:2
- Mate:21: frame_1385mm:2 ↔ frame_215.5mm:5
- Flush:32: frame_1385mm:2 ↔ frame_215.5mm:5
- Flush:33 (110 mm): frame_1385mm:2 ↔ frame_215.5mm:5
- Mate:22: frame_1385mm:1 ↔ frame_215.5mm:8
- Flush:34: frame_1385mm:1 ↔ frame_215.5mm:8
- Flush:35: frame_215.5mm:5 ↔ frame_215.5mm:8
- Mate:23: frame_1385mm:1 ↔ frame_215.5mm:9
- Flush:36: frame_1385mm:1 ↔ frame_215.5mm:9
- Flush:37: frame_265mm:4 ↔ frame_215.5mm:9
- Mate:24: frame_1385mm:1 ↔ frame_215.5mm:7
- Flush:38: frame_1385mm:1 ↔ frame_215.5mm:7
- Flush:39: frame_265mm:5 ↔ frame_215.5mm:7
- Mate:25: frame_265mm:6 ↔ frame_215.5mm:6
- Flush:40: frame_265mm:6 ↔ frame_215.5mm:6
- Flush:41: frame_265mm:6 ↔ frame_215.5mm:6
- Mate:26: frame_265mm:6 ↔ frame_215.5mm:10
- Flush:42: frame_265mm:5 ↔ frame_215.5mm:10
- Flush:43: frame_265mm:6 ↔ frame_215.5mm:10
- Mate:27: frame_215.5mm:5 ↔ frame_1385mm:3
- Flush:44: frame_1385mm:2 ↔ frame_1385mm:3
- Flush:45: frame_1385mm:2 ↔ frame_1385mm:3
- Mate:28: frame_215.5mm:8 ↔ frame_1385mm:4
- Flush:46: frame_1385mm:1 ↔ frame_1385mm:4
- Flush:47: frame_1385mm:1 ↔ frame_1385mm:4
- Mate:29: frame_215.5mm:6 ↔ frame_265mm:7
- Flush:48: frame_215.5mm:6 ↔ frame_265mm:7
- Flush:49: frame_215.5mm:6 ↔ frame_265mm:7
- Mate:30: frame_1385mm:4 ↔ frame_265mm:10
- Flush:50: frame_265mm:7 ↔ frame_265mm:10
- Flush:51: frame_265mm:7 ↔ frame_265mm:10
- Mate:31: frame_1385mm:4 ↔ frame_265mm:8
- Flush:52: frame_265mm:7 ↔ frame_265mm:8
- Flush:53: frame_265mm:7 ↔ frame_265mm:8
- Mate:32: frame_215.5mm:4 ↔ frame_265mm:9
- Flush:54: frame_215.5mm:4 ↔ frame_265mm:9
- Flush:55: frame_215.5mm:4 ↔ frame_265mm:9
- Mate:33: frame_1385mm:3 ↔ frame_265mm:12
- Flush:56: frame_265mm:9 ↔ frame_265mm:12
- Flush:57: frame_265mm:9 ↔ frame_265mm:12
- Mate:34: frame_1385mm:3 ↔ frame_265mm:11
- Flush:58: frame_265mm:9 ↔ frame_265mm:11
- Flush:59: frame_265mm:9 ↔ frame_265mm:11
- Mate:35: frame_1385mm:4 ↔ frame_300mm:4
- Flush:60: frame_1385mm:4 ↔ frame_300mm:4
- Flush:61: frame_300mm:2 ↔ frame_300mm:4
- Mate:36: frame_1385mm:4 ↔ frame_300mm:5
- Flush:62: frame_1385mm:4 ↔ frame_300mm:5
- Flush:63: frame_300mm:3 ↔ frame_300mm:5
- Flush:66: frame_1660mm:2 ↔ frame_1660mm:3
- Flush:67: frame_1385mm:1 ↔ frame_1660mm:3
- Mate:38 (-45 mm): frame_1385mm:1 ↔ frame_1660mm:3
- Mate:39: frame_1385mm:1 ↔ frame_1660mm:3
- Mate:40: frame_210mm:1 ↔ frame_1660mm:3
- Flush:68: frame_210mm:1 ↔ frame_1660mm:3
- Flush:69: frame_210mm:1 ↔ frame_1660mm:3
- Mate:42: frame_210mm:2 ↔ frame_1660mm:3
- Flush:72: frame_210mm:2 ↔ frame_1660mm:3
- Mate:43 (100 mm): frame_210mm:1 ↔ frame_210mm:2
- Mate:44: frame_210mm:3 ↔ frame_1660mm:3
- Flush:73: frame_210mm:3 ↔ frame_1660mm:3
- Flush:74 (670 mm): frame_1660mm:2 ↔ frame_210mm:3
- Mate:45: frame_210mm:4 ↔ frame_1660mm:3
- Flush:75: frame_210mm:4 ↔ frame_1660mm:3
- Flush:76 (1325 mm): frame_210mm:1 ↔ frame_210mm:4
- Mate:46: 1222_Former Shaft Plate_V1:1 ↔ frame_300mm:2
- Flush:77: 1222_Former Shaft Plate_V1:1 ↔ frame_300mm:2
- Mate:47 (126 mm): 1222_Former Shaft Plate_V1:1 ↔ frame_1385mm:2
- Mate:48: 1222_Former Shaft Plate_V1:2 ↔ frame_300mm:4
- Flush:78: 1222_Former Shaft Plate_V1:2 ↔ frame_300mm:4
- Mate:49 (126 mm): 1222_Former Shaft Plate_V1:2 ↔ frame_1385mm:3
- Insert:1 (-45 mm): 1222_Former Shaft Plate_V1:1 ↔ 1221_Center Former Shaft_V1:1
- Mate:50: 1228_Major Gear_V1:1 ↔ frame_1385mm:4
- Mate:51: 1221_Center Former Shaft_V1:1 ↔ 1228_Major Gear_V1:1
- Insert:2: 1228_Major Gear_V1:1 ↔ 1227_Former Shaft Bearing_V1:1
- Mate:52: 1228_Major Gear_V1:1 ↔ 1313_Former Bottom_V1:1
- Mate:53: 1221_Center Former Shaft_V1:1 ↔ 1313_Former Bottom_V1:1
- Insert:3: 1228_Major Gear_V1:1 ↔ 1313_Former Bottom_V1:1
- Insert:4: 1228_Major Gear_V1:1 ↔ 1313_Former Bottom_V1:1
- Insert:5: 1228_Major Gear_V1:1 ↔ 1226_Flat Head Screw_V1:8
- Insert:6: 1228_Major Gear_V1:1 ↔ 1226_Flat Head Screw_V1:12
- Insert:7: 1228_Major Gear_V1:1 ↔ 1226_Flat Head Screw_V1:4
- Insert:8: 1228_Major Gear_V1:1 ↔ 1226_Flat Head Screw_V1:11
- Insert:9: 1228_Major Gear_V1:1 ↔ 1226_Flat Head Screw_V1:10
- Insert:10: 1228_Major Gear_V1:1 ↔ 1226_Flat Head Screw_V1:1
- Insert:11: 1228_Major Gear_V1:1 ↔ 1226_Flat Head Screw_V1:5
- Insert:12: 1228_Major Gear_V1:1 ↔ 1226_Flat Head Screw_V1:6
- Insert:13: 1228_Major Gear_V1:1 ↔ 1226_Flat Head Screw_V1:7
- Insert:14: 1228_Major Gear_V1:1 ↔ 1226_Flat Head Screw_V1:2
- Insert:15: 1228_Major Gear_V1:1 ↔ 1226_Flat Head Screw_V1:3
- Insert:16: 1228_Major Gear_V1:1 ↔ 1226_Flat Head Screw_V1:9
- Mate:54: 1313_Former Bottom_V1:1 ↔ 1312_Former Middle_V1:1
- Mate:55: 1221_Center Former Shaft_V1:1 ↔ 1312_Former Middle_V1:1
- Insert:17: 1313_Former Bottom_V1:1 ↔ 1312_Former Middle_V1:1
- Mate:56: 1312_Former Middle_V1:1 ↔ 1311_Former Top_V1:1
- Mate:57: 1221_Center Former Shaft_V1:1 ↔ 1311_Former Top_V1:1
- Insert:18: 1312_Former Middle_V1:1 ↔ 1311_Former Top_V1:1
- Mate:58: 1311_Former Top_V1:1 ↔ 1324_Clamp Rail_V1:1
- Insert:31: 1311_Former Top_V1:1 ↔ 1324_Clamp Rail_V1:1
- Insert:32: 1311_Former Top_V1:1 ↔ 1324_Clamp Rail_V1:1
- Mate:59: 1311_Former Top_V1:1 ↔ 1324_Clamp Rail_V1:2
- Insert:33: 1311_Former Top_V1:1 ↔ 1324_Clamp Rail_V1:2
- Insert:34: 1311_Former Top_V1:1 ↔ 1324_Clamp Rail_V1:2
- Mate:60: 1311_Former Top_V1:1 ↔ 1322_Clamp Holder_V1:1
- Flush:79 (45 mm): 1324_Clamp Rail_V1:1 ↔ 1322_Clamp Holder_V1:1
- Mate:61 (0.5 mm): 1324_Clamp Rail_V1:2 ↔ 1322_Clamp Holder_V1:1
- Mate:62: 1322_Clamp Holder_V1:1 ↔ 1321_Toggle Clamp_V1:1
- Flush:80: 1322_Clamp Holder_V1:1 ↔ 1321_Toggle Clamp_V1:1
- Flush:81 (3 mm): 1322_Clamp Holder_V1:1 ↔ 1321_Toggle Clamp_V1:1
- Insert:35: 1311_Former Top_V1:1 ↔ 1323_Clamp Holder Pin_V1:1
- Insert:36: 1311_Former Top_V1:1 ↔ 1326_Thumb Screw_V1:2
- Insert:37: 1311_Former Top_V1:1 ↔ 1326_Thumb Screw_V1:1
- Mate:63: frame_1385mm:3 ↔ 1223_Motor Plate_V1:1
- Flush:82: frame_1385mm:3 ↔ 1223_Motor Plate_V1:1
- Flush:83: frame_1385mm:3 ↔ 1223_Motor Plate_V1:1
- Insert:38: 1224a_Stepper Motor Gearbox_V1:1 ↔ 1223_Motor Plate_V1:1
- Insert:39: 1224a_Stepper Motor Gearbox_V1:1 ↔ 1223_Motor Plate_V1:1
- Insert:40: 1224a_Stepper Motor Gearbox_V1:1 ↔ 1224_Stepper Motor_V1:1
- Insert:41: 1224a_Stepper Motor Gearbox_V1:1 ↔ 1224_Stepper Motor_V1:1
- Flush:84: 1228_Major Gear_V1:1 ↔ 1225_Pinon_V1:1
- Mate:64: 1225_Pinon_V1:1 ↔ 1225a_Pinion Collar_V1:1
- Mate:65: 1224a_Stepper Motor Gearbox_V1:1 ↔ 1225a_Pinion Collar_V1:1
- Insert:42: 1225_Pinon_V1:1 ↔ 1225a_Pinion Collar_V1:1
- Insert:43: 1225_Pinon_V1:1 ↔ 1225a_Pinion Collar_V1:1
- Insert:44: 1213_Distal Roller_V1:1 ↔ 12114_3-8 Shaft Bearing_V1:1
- Insert:45: 1213_Distal Roller_V1:2 ↔ 12114_3-8 Shaft Bearing_V1:2
- Insert:46 (0.5 mm): 1211_Distal Roller Plate_V1:1 ↔ 1213_Distal Roller_V1:1
- Insert:47 (0.5 mm): 1211_Distal Roller Plate_V1:1 ↔ 1213_Distal Roller_V1:2
- Insert:48: 1213_Distal Roller_V1:1 ↔ 12114_3-8 Shaft Bearing_V1:3
- Insert:49: 1213_Distal Roller_V1:2 ↔ 12114_3-8 Shaft Bearing_V1:4
- Mate:68 (0.5 mm): 1213_Distal Roller_V1:2 ↔ 1211_Distal Roller Plate_V1:2
- Flush:87: 1211_Distal Roller Plate_V1:1 ↔ 1211_Distal Roller Plate_V1:2
- Flush:88: 1211_Distal Roller Plate_V1:1 ↔ 1211_Distal Roller Plate_V1:2
- Insert:50: 1211_Distal Roller Plate_V1:1 ↔ 1216_Roller Spacer_V1:2
- Insert:51: 1211_Distal Roller Plate_V1:1 ↔ 1216_Roller Spacer_V1:1
- Insert:52: 1211_Distal Roller Plate_V1:2 ↔ 1212_Roller Plate Bolt_V1:1
- Insert:53: 1211_Distal Roller Plate_V1:2 ↔ 1212_Roller Plate Bolt_V1:2
- Insert:54 (-14 mm): 1211_Distal Roller Plate_V1:2 ↔ 1215_3-8 Roller Shaft_V1:1
- Insert:55 (-14 mm): 1211_Distal Roller Plate_V1:2 ↔ 1215_3-8 Roller Shaft_V1:2
- Insert:56: 1211_Distal Roller Plate_V1:2 ↔ 1214_Shaft Collar 3-16_V1:3
- Insert:57: 1211_Distal Roller Plate_V1:2 ↔ 1214_Shaft Collar 3-16_V1:4
- Insert:58: 1211_Distal Roller Plate_V1:1 ↔ 1214_Shaft Collar 3-16_V1:1
- Insert:59: 1211_Distal Roller Plate_V1:1 ↔ 1214_Shaft Collar 3-16_V1:2
- Mate:69: frame_275mm:1 ↔ frame_1660mm:2
- Mate:70: 1211_Distal Roller Plate_V1:1 ↔ frame_275mm:1
- Flush:89: frame_275mm:1 ↔ frame_210mm:1
- Flush:90: frame_275mm:1 ↔ frame_1660mm:2
- Mate:71: frame_275mm:2 ↔ frame_1660mm:3
- Mate:72: 1211_Distal Roller Plate_V1:1 ↔ frame_275mm:2
- Flush:91: frame_275mm:2 ↔ frame_210mm:1
- Flush:92: frame_275mm:2 ↔ frame_1660mm:3
- Mate:73: frame_318mm:1 ↔ frame_1660mm:3
- Flush:93: frame_318mm:1 ↔ frame_210mm:2
- Flush:94: frame_318mm:1 ↔ frame_1660mm:3
- Mate:74: frame_318mm:2 ↔ frame_1660mm:2
- Flush:95: frame_318mm:2 ↔ frame_210mm:2
- Flush:96: frame_318mm:2 ↔ frame_1660mm:2
- Mate:75: 12110_Shaft Cap_V1:1 ↔ frame_318mm:2
- Mate:76: 12110_Shaft Cap_V1:1 ↔ frame_318mm:2
- Mate:77: 12110_Shaft Cap_V1:1 ↔ frame_318mm:2
- Mate:78: 12110_Shaft Cap_V1:2 ↔ frame_318mm:1
- Mate:79: 12110_Shaft Cap_V1:2 ↔ frame_318mm:1
- Mate:80: 12110_Shaft Cap_V1:2 ↔ frame_318mm:1
- Insert:60 (-10 mm): 12110_Shaft Cap_V1:2 ↔ 1217_17mm Shaft_V1:1
- Insert:61 (44 mm): 12110_Shaft Cap_V1:2 ↔ 1219_Middle Roller_V1:1
- Insert:62: 1219_Middle Roller_V1:1 ↔ 1218_Angular Contact Bearing 17mm_V1:1
- Insert:63: 1219_Middle Roller_V1:1 ↔ 1218_Angular Contact Bearing 17mm_V1:2
- Mate:81: frame_440mm:1 ↔ frame_1660mm:3
- Flush:97: frame_440mm:1 ↔ frame_1660mm:3
- Flush:98: frame_440mm:1 ↔ frame_210mm:3
- Mate:82: frame_440mm:2 ↔ frame_1660mm:2
- Flush:99: frame_440mm:2 ↔ frame_1660mm:2
- Flush:100: frame_440mm:2 ↔ frame_210mm:3
- Mate:83: frame_440mm:2 ↔ 12112_Proximal Roller Plate_V1:1
- Flush:101 (8.5 mm): frame_440mm:2 ↔ 12112_Proximal Roller Plate_V1:1
- Flush:102 (10 mm): frame_440mm:2 ↔ 12112_Proximal Roller Plate_V1:1
- Mate:84: frame_440mm:1 ↔ 12112_Proximal Roller Plate_V1:2
- Flush:103 (10 mm): frame_440mm:1 ↔ 12112_Proximal Roller Plate_V1:2
- Flush:104 (8.5 mm): frame_440mm:1 ↔ 12112_Proximal Roller Plate_V1:2
- Insert:64 (2 mm): 12112_Proximal Roller Plate_V1:2 ↔ 12113_Proximal Roller Shaft_V1:1
- Insert:65 (2 mm): 12112_Proximal Roller Plate_V1:2 ↔ 12113_Proximal Roller Shaft_V1:2
- Insert:66: 12111_Proximal Roller_V1:1 ↔ 12114_3-8 Shaft Bearing_V1:5
- Insert:67: 12111_Proximal Roller_V1:2 ↔ 12114_3-8 Shaft Bearing_V1:7
- Insert:68: 12111_Proximal Roller_V1:1 ↔ 12114_3-8 Shaft Bearing_V1:6
- Insert:69: 12111_Proximal Roller_V1:2 ↔ 12114_3-8 Shaft Bearing_V1:8
- Insert:70 (5 mm): 12112_Proximal Roller Plate_V1:2 ↔ 12111_Proximal Roller_V1:1
- Insert:71 (5 mm): 12112_Proximal Roller Plate_V1:2 ↔ 12111_Proximal Roller_V1:2
- Flush:105: frame_370mm:3 ↔ frame_1660mm:3
- Flush:106: frame_370mm:3 ↔ frame_1660mm:3
- Mate:85: frame_370mm:3 ↔ frame_1660mm:3
- Flush:107: frame_370mm:4 ↔ frame_1660mm:3
- Mate:86: frame_370mm:4 ↔ frame_1660mm:3
- Mate:87: frame_370mm:1 ↔ frame_1660mm:2
- Mate:88: frame_370mm:2 ↔ frame_1660mm:2
- Flush:108: frame_370mm:1 ↔ frame_1660mm:2
- Flush:109: frame_370mm:1 ↔ frame_1660mm:2
- Flush:110: frame_370mm:2 ↔ frame_1660mm:2
- Mate:89: 1236_Spool Shaft Support Plate_V1:2 ↔ frame_370mm:1
- Flush:111: 1236_Spool Shaft Support Plate_V1:2 ↔ frame_370mm:1
- Flush:112: 1236_Spool Shaft Support Plate_V1:2 ↔ frame_370mm:1
- Flush:113: 1236_Spool Shaft Support Plate_V1:2 ↔ frame_370mm:2
- Insert:72: 12112_Proximal Roller Plate_V1:2 ↔ 92991A190_BRASS CUP POINT SET SCREW:2
- Insert:73: 12112_Proximal Roller Plate_V1:2 ↔ 92991A190_BRASS CUP POINT SET SCREW:1
- Insert:74: 12112_Proximal Roller Plate_V1:1 ↔ 92991A190_BRASS CUP POINT SET SCREW:4
- Insert:75: 12112_Proximal Roller Plate_V1:1 ↔ 92991A190_BRASS CUP POINT SET SCREW:3
- Mate:90: 1236_Spool Shaft Support Plate_V1:1 ↔ frame_370mm:3
- Flush:114: 1236_Spool Shaft Support Plate_V1:1 ↔ frame_370mm:3
- Flush:115: 1236_Spool Shaft Support Plate_V1:1 ↔ frame_370mm:3
- Flush:116: 1236_Spool Shaft Support Plate_V1:1 ↔ frame_370mm:4
- Insert:76 (-26 mm): 1236_Spool Shaft Support Plate_V1:1 ↔ 1231_Spool Shaft_V1:1
- Insert:77: 1236_Spool Shaft Support Plate_V1:1 ↔ 1232_Spool Shaft Collar_V1:1
- Insert:78: 1236_Spool Shaft Support Plate_V1:2 ↔ 1232_Spool Shaft Collar_V1:2
- Angle:1 (0 deg): 1236_Spool Shaft Support Plate_V1:2 ↔ 1231_Spool Shaft_V1:1
- Insert:82: 1234_Spool Plate_V1:2 ↔ 1233_Spool Holding Bolts_V1:1
- Insert:83: 1234_Spool Plate_V1:2 ↔ 1233_Spool Holding Bolts_V1:2
- Insert:84: 1234_Spool Plate_V1:1 ↔ 1233_Spool Holding Bolts_V1:3
- Insert:85: 1234_Spool Plate_V1:1 ↔ 1233_Spool Holding Bolts_V1:4
- Insert:86: 1234_Spool Plate_V1:1 ↔ 1235_Shaft Locking Screw_V1:1
- Insert:87: 1234_Spool Plate_V1:2 ↔ 1235_Shaft Locking Screw_V1:2
- Insert:88 (5 mm): 12310_Washer_V1:1 ↔ frame_1660mm:2
- Insert:89 (5 mm): 12310_Washer_V1:2 ↔ frame_1660mm:3
- Insert:90: 12310_Washer_V1:2 ↔ 1239_Turnbuckle Holding Bolt_V1:2
- Insert:91: 12310_Washer_V1:1 ↔ 1239_Turnbuckle Holding Bolt_V1:1
- Insert:92 (5 mm): 12310_Washer_V1:3 ↔ frame_1660mm:2
- Insert:93 (5 mm): 12310_Washer_V1:4 ↔ frame_1660mm:3
- Insert:94: 12310_Washer_V1:4 ↔ 1238_Hex Nut Turnbuckle_V1:1
- Insert:95: 1238_Hex Nut Turnbuckle_V1:1 ↔ 1238_Hex Nut Turnbuckle_V1:2
- Insert:96: 12310_Washer_V1:3 ↔ 1238_Hex Nut Turnbuckle_V1:3
- Insert:97: 1238_Hex Nut Turnbuckle_V1:3 ↔ 1238_Hex Nut Turnbuckle_V1:4
- Mate:91: 1239_Turnbuckle Holding Bolt_V1:1 ↔ 1237_Turnbuckle_V1:1
- Angle:3 (0 deg): 1237_Turnbuckle_V1:1 ↔ frame_370mm:2
- Mate:92: 1239_Turnbuckle Holding Bolt_V1:2 ↔ 1237_Turnbuckle_V1:2
- Angle:4 (0 deg): 1237_Turnbuckle_V1:2 ↔ frame_370mm:4
- Insert:98 (2 mm): 1239_Turnbuckle Holding Bolt_V1:1 ↔ 1238_Hex Nut Turnbuckle_V1:5
- Insert:99 (8 mm): 1239_Turnbuckle Holding Bolt_V1:2 ↔ 1238_Hex Nut Turnbuckle_V1:6
- Insert:100: 1325_Former Plate Bolts_V1:1 ↔ 1311_Former Top_V1:1
- Insert:101: 1325_Former Plate Bolts_V1:2 ↔ 1311_Former Top_V1:1
- Insert:102: 1325_Former Plate Bolts_V1:3 ↔ 1311_Former Top_V1:1
- Insert:103: 1325_Former Plate Bolts_V1:4 ↔ 1311_Former Top_V1:1
- Insert:104: 1325_Former Plate Bolts_V1:5 ↔ 1311_Former Top_V1:1
- Insert:105: 1325_Former Plate Bolts_V1:6 ↔ 1311_Former Top_V1:1
- Insert:106: 1325_Former Plate Bolts_V1:7 ↔ 1311_Former Top_V1:1
- Insert:107: 1325_Former Plate Bolts_V1:8 ↔ 1311_Former Top_V1:1
- Insert:108: 1325_Former Plate Bolts_V1:9 ↔ 1311_Former Top_V1:1
- Insert:109: 1325_Former Plate Bolts_V1:10 ↔ 1311_Former Top_V1:1
- Insert:110: 1325_Former Plate Bolts_V1:11 ↔ 1311_Former Top_V1:1
- Insert:111: 1325_Former Plate Bolts_V1:12 ↔ 1311_Former Top_V1:1
- Mate:93: 1322_Clamp Holder_V1:1 ↔ BS 3692 Precision hexagon bolts and screws (Full Threaded) - Metric M4 x 9:2
- Mate:94: 1322_Clamp Holder_V1:1 ↔ BS 3692 Precision hexagon bolts and screws (Full Threaded) - Metric M4 x 9:2
- Angle:5 (0 deg): 1322_Clamp Holder_V1:1 ↔ BS 3692 Precision hexagon bolts and screws (Full Threaded) - Metric M4 x 9:2
- Mate:95: 1322_Clamp Holder_V1:1 ↔ BS 3692 Precision hexagon bolts and screws (Full Threaded) - Metric M4 x 9:1
- Mate:96: 1322_Clamp Holder_V1:1 ↔ BS 3692 Precision hexagon bolts and screws (Full Threaded) - Metric M4 x 9:1
- Angle:6 (0 deg): 1322_Clamp Holder_V1:1 ↔ BS 3692 Precision hexagon bolts and screws (Full Threaded) - Metric M4 x 9:1
- Flush:118: BS 3692 Precision hexagon bolts and screws (Full Threaded) - Metric M4 x 9:3 ↔ BS 3692 Precision hexagon bolts and screws (Full Threaded) - Metric M4 x 9:4
- Mate:97: 1322_Clamp Holder_V1:1 ↔ BS 3692 Precision hexagon bolts and screws (Full Threaded) - Metric M4 x 9:4
- Mate:98: 1322_Clamp Holder_V1:1 ↔ BS 3692 Precision hexagon bolts and screws (Full Threaded) - Metric M4 x 9:4
- Flush:119: BS 3692 Precision hexagon bolts and screws (Full Threaded) - Metric M4 x 9:1 ↔ BS 3692 Precision hexagon bolts and screws (Full Threaded) - Metric M4 x 9:4
- Mate:99: 1322_Clamp Holder_V1:1 ↔ BS 3692 Precision hexagon bolts and screws (Full Threaded) - Metric M4 x 9:3
- Flush:120: BS 3692 Precision hexagon bolts and screws (Full Threaded) - Metric M4 x 9:2 ↔ BS 3692 Precision hexagon bolts and screws (Full Threaded) - Metric M4 x 9:3
- Mate:100: BS 3692 Precision hexagon bolts and screws (Full Threaded) - Metric M4 x 9:1 ↔ AS 1474 - Metric M4:1
- Mate:101: 1321_Toggle Clamp_V1:1 ↔ AS 1474 - Metric M4:1
- Flush:121: AS 1474 - Metric M4:2 ↔ AS 1474 - Metric M4:4
- Flush:122: AS 1474 - Metric M4:3 ↔ AS 1474 - Metric M4:4
- Flush:123: AS 1474 - Metric M4:2 ↔ AS 1474 - Metric M4:3
- Mate:102: BS 3692 Precision hexagon bolts and screws (Full Threaded) - Metric M4 x 9:4 ↔ AS 1474 - Metric M4:2
- Mate:103: 1321_Toggle Clamp_V1:1 ↔ AS 1474 - Metric M4:2
- Mate:104: BS 3692 Precision hexagon bolts and screws (Full Threaded) - Metric M4 x 9:3 ↔ AS 1474 - Metric M4:3
- Mate:105: 1321_Toggle Clamp_V1:1 ↔ AS 1474 - Metric M4:4
- Mate:106: BS 3692 Precision hexagon bolts and screws (Full Threaded) - Metric M4 x 9:2 ↔ AS 1474 - Metric M4:4
- Flush:124: AS 1474 - Metric M4:1 ↔ AS 1474 - Metric M4:4
- [Mate]: 1322_Clamp Holder_V1:2 ↔ 1321_Toggle Clamp_V1:2
- [Flush]: 1322_Clamp Holder_V1:2 ↔ 1321_Toggle Clamp_V1:2
- [Flush] (3 mm): 1322_Clamp Holder_V1:2 ↔ 1321_Toggle Clamp_V1:2
- [Mate]: 1322_Clamp Holder_V1:2 ↔ BS 3692 Precision hexagon bolts and screws (Full Threaded) - Metric M4 x 9:6
- [Mate]: 1322_Clamp Holder_V1:2 ↔ BS 3692 Precision hexagon bolts and screws (Full Threaded) - Metric M4 x 9:6
- [Angle] (0 deg): 1322_Clamp Holder_V1:2 ↔ BS 3692 Precision hexagon bolts and screws (Full Threaded) - Metric M4 x 9:6
- [Mate]: 1322_Clamp Holder_V1:2 ↔ BS 3692 Precision hexagon bolts and screws (Full Threaded) - Metric M4 x 9:5
- [Mate]: 1322_Clamp Holder_V1:2 ↔ BS 3692 Precision hexagon bolts and screws (Full Threaded) - Metric M4 x 9:5
- [Angle] (0 deg): 1322_Clamp Holder_V1:2 ↔ BS 3692 Precision hexagon bolts and screws (Full Threaded) - Metric M4 x 9:5
- [Flush]: BS 3692 Precision hexagon bolts and screws (Full Threaded) - Metric M4 x 9:7 ↔ BS 3692 Precision hexagon bolts and screws (Full Threaded) - Metric M4 x 9:8
- [Mate]: 1322_Clamp Holder_V1:2 ↔ BS 3692 Precision hexagon bolts and screws (Full Threaded) - Metric M4 x 9:8
- [Mate]: 1322_Clamp Holder_V1:2 ↔ BS 3692 Precision hexagon bolts and screws (Full Threaded) - Metric M4 x 9:8
- [Flush]: BS 3692 Precision hexagon bolts and screws (Full Threaded) - Metric M4 x 9:5 ↔ BS 3692 Precision hexagon bolts and screws (Full Threaded) - Metric M4 x 9:8
- [Mate]: 1322_Clamp Holder_V1:2 ↔ BS 3692 Precision hexagon bolts and screws (Full Threaded) - Metric M4 x 9:7
- [Flush]: BS 3692 Precision hexagon bolts and screws (Full Threaded) - Metric M4 x 9:6 ↔ BS 3692 Precision hexagon bolts and screws (Full Threaded) - Metric M4 x 9:7
- [Mate]: BS 3692 Precision hexagon bolts and screws (Full Threaded) - Metric M4 x 9:5 ↔ AS 1474 - Metric M4:5
- [Mate]: 1321_Toggle Clamp_V1:2 ↔ AS 1474 - Metric M4:5
- [Flush]: AS 1474 - Metric M4:6 ↔ AS 1474 - Metric M4:8
- [Flush]: AS 1474 - Metric M4:7 ↔ AS 1474 - Metric M4:8
- [Flush]: AS 1474 - Metric M4:6 ↔ AS 1474 - Metric M4:7
- [Mate]: BS 3692 Precision hexagon bolts and screws (Full Threaded) - Metric M4 x 9:8 ↔ AS 1474 - Metric M4:6
- [Mate]: 1321_Toggle Clamp_V1:2 ↔ AS 1474 - Metric M4:6
- [Mate]: BS 3692 Precision hexagon bolts and screws (Full Threaded) - Metric M4 x 9:7 ↔ AS 1474 - Metric M4:7
- [Mate]: 1321_Toggle Clamp_V1:2 ↔ AS 1474 - Metric M4:8
- [Mate]: BS 3692 Precision hexagon bolts and screws (Full Threaded) - Metric M4 x 9:6 ↔ AS 1474 - Metric M4:8
- [Flush]: AS 1474 - Metric M4:5 ↔ AS 1474 - Metric M4:8
- Mate:122: 1311_Former Top_V1:1 ↔ 1322_Clamp Holder_V1:2
- Flush:134: 1311_Former Top_V1:1 ↔ 1323_Clamp Holder Pin_V1:2
- Mate:123: 1324_Clamp Rail_V1:2 ↔ 1322_Clamp Holder_V1:2